# Autodesk Inventor assembly: First Iteration Intake
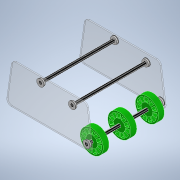
[picture p0: Inventor's stored thumbnail of the model, 180x180]
Saved by Autodesk Inventor 2021 (Build 250183000, 183)
## iProperties
Created: 2021-01-29
Part Number: First Iteration Intake
Document SubType Name: Assembly
Designer: aidan
Author: aidan
## Documents named in this file (5)
- C:\Users\aidan\Desktop\T3 Robotics\CAD\2021 Specific Parts\First Iteration Intake.iam
- C:\Users\aidan\Desktop\T3 Robotics\CAD\16in THUNDERSHAFT.ipt
- C:\Users\aidan\Desktop\T3 Robotics\CAD\Tony's CAD\Compliance wheel.ipt
- C:\Users\aidan\Desktop\T3 Robotics\CAD\2021 Specific Parts\2021 Intake Panels.ipt
- C:\Users\aidan\Desktop\T3 Robotics\CAD\Bearing for THUNDER.ipt
## Components (14 placed, 4 different names)
1. 16in THUNDERSHAFT:1 — Mate:11, Flush:11, Flush:12
2. 16in THUNDERSHAFT:2 — Mate:13, Flush:10, Flush:11, Flush:13
3. 16in THUNDERSHAFT:3 — Mate:1, Mate:2, Mate:14, Flush:10
4. Compliance wheel:1 — Flush:1, Flush:3, Mate:1, Mate:2
5. Compliance wheel:2 — Flush:1, Flush:2, Flush:3, Flush:4
6. Compliance wheel:3 — Flush:2, Flush:4
7. 2021 Intake Panels:1 — Mate:4, Mate:5, Mate:6, Mate:7, Flush:9
8. 2021 Intake Panels:2 — Mate:3, Mate:8, Mate:9, Mate:10, Flush:9
9. Bearing for THUNDER:1 — Flush:5, Mate:5, Mate:11, Mate:12, Flush:12
10. Bearing for THUNDER:2 — Flush:5, Flush:6, Mate:4, Mate:6, Mate:13
11. Bearing for THUNDER:3 — Flush:6, Mate:7, Mate:14
12. Bearing for THUNDER:4 — Flush:7, Mate:10, Mate:12
13. Bearing for THUNDER:5 — Flush:7, Flush:8, Mate:3, Mate:9, Flush:13
14. Bearing for THUNDER:6 — Flush:8, Mate:8
## Relationships (27: Mate 14, Flush 13)
- Flush:1: Compliance wheel:1 ↔ Compliance wheel:2
- Flush:2: Compliance wheel:2 ↔ Compliance wheel:3
- Flush:3: Compliance wheel:1 ↔ Compliance wheel:2
- Flush:4: Compliance wheel:2 ↔ Compliance wheel:3
- Mate:1: 16in THUNDERSHAFT:3 ↔ Compliance wheel:1
- Mate:2: 16in THUNDERSHAFT:3 ↔ Compliance wheel:1
- Flush:5: Bearing for THUNDER:1 ↔ Bearing for THUNDER:2
- Flush:6: Bearing for THUNDER:2 ↔ Bearing for THUNDER:3
- Flush:7: Bearing for THUNDER:4 ↔ Bearing for THUNDER:5
- Flush:8: Bearing for THUNDER:5 ↔ Bearing for THUNDER:6
- Mate:3: 2021 Intake Panels:2 ↔ Bearing for THUNDER:5
- Mate:4: 2021 Intake Panels:1 ↔ Bearing for THUNDER:2
- Mate:5: 2021 Intake Panels:1 ↔ Bearing for THUNDER:1
- Mate:6: 2021 Intake Panels:1 ↔ Bearing for THUNDER:2
- Mate:7: 2021 Intake Panels:1 ↔ Bearing for THUNDER:3
- Mate:8: 2021 Intake Panels:2 ↔ Bearing for THUNDER:6
- Mate:9: 2021 Intake Panels:2 ↔ Bearing for THUNDER:5
- Mate:10: 2021 Intake Panels:2 ↔ Bearing for THUNDER:4
- Flush:9: 2021 Intake Panels:1 ↔ 2021 Intake Panels:2
- Mate:11: 16in THUNDERSHAFT:1 ↔ Bearing for THUNDER:1
- Mate:12: Bearing for THUNDER:1 ↔ Bearing for THUNDER:4
- Mate:13: 16in THUNDERSHAFT:2 ↔ Bearing for THUNDER:2
- Mate:14: 16in THUNDERSHAFT:3 ↔ Bearing for THUNDER:3
- Flush:10: 16in THUNDERSHAFT:2 ↔ 16in THUNDERSHAFT:3
- Flush:11: 16in THUNDERSHAFT:1 ↔ 16in THUNDERSHAFT:2
- Flush:12: 16in THUNDERSHAFT:1 ↔ Bearing for THUNDER:1
- Flush:13: 16in THUNDERSHAFT:2 ↔ Bearing for THUNDER:5
